# Autodesk Inventor assembly: printer
(part 3 of 3)
- Mate:775: CSN 02 1702 B B 4,3:170 ↔ ISO 4762 M4 x 20:78
- Mate:776: CSN 02 1702 B B 4,3:169 ↔ ISO 4762 M4 x 20:79
- Mate:777: CSN 02 1702 B B 4,3:167 ↔ ISO 4762 M4 x 20:81
- Mate:778: CSN 02 1702 B B 4,3:168 ↔ ISO 4762 M4 x 20:80
- Mate:779: CSN 02 1702 B B 4,3:171 ↔ DIN EN ISO 7040 M4:83
- Mate:780: ISO 4762 M4 x 20:77 ↔ DIN EN ISO 7040 M4:83
- Mate:781: CSN 02 1702 B B 4,3:172 ↔ DIN EN ISO 7040 M4:82
- Mate:782: ISO 4762 M4 x 20:76 ↔ DIN EN ISO 7040 M4:82
- Mate:783: CSN 02 1702 B B 4,3:173 ↔ DIN EN ISO 7040 M4:81
- Mate:784: ISO 4762 M4 x 20:75 ↔ DIN EN ISO 7040 M4:81
- Mate:785: CSN 02 1702 B B 4,3:174 ↔ DIN EN ISO 7040 M4:80
- Mate:786: ISO 4762 M4 x 20:74 ↔ DIN EN ISO 7040 M4:80
- Mate:787: CSN 02 1702 B B 4,3:170 ↔ DIN EN ISO 7040 M4:84
- Mate:788: ISO 4762 M4 x 20:78 ↔ DIN EN ISO 7040 M4:84
- Mate:789: CSN 02 1702 B B 4,3:169 ↔ DIN EN ISO 7040 M4:87
- Mate:790: ISO 4762 M4 x 20:79 ↔ DIN EN ISO 7040 M4:87
- Mate:791: CSN 02 1702 B B 4,3:168 ↔ DIN EN ISO 7040 M4:86
- Mate:792: ISO 4762 M4 x 20:80 ↔ DIN EN ISO 7040 M4:86
- Mate:793: CSN 02 1702 B B 4,3:167 ↔ DIN EN ISO 7040 M4:85
- Mate:794: ISO 4762 M4 x 20:81 ↔ DIN EN ISO 7040 M4:85
- Mate:795: brace_right:1 ↔ IEC inlet:1
- Mate:796: brace_right:1 ↔ IEC inlet:1
- Mate:797: brace_right:1 ↔ IEC inlet:1
- Insert:159: IEC inlet:1 ↔ Cross Recessed Flat Countersunk Head Tapping Screw - Type AB - Type IA - Metric 2,9 x 1 x 8:1
- Insert:160: IEC inlet:1 ↔ Cross Recessed Flat Countersunk Head Tapping Screw - Type AB - Type IA - Metric 2,9 x 1 x 8:2
- Mate:801: back:1 ↔ PC Fan:1
- Mate:802: back:1 ↔ PC Fan:1
- Mate:803: back:1 ↔ PC Fan:1
- Mate:804 (3 mm): back:1 ↔ User Library-Fan Guard:1
- Tangent:3: back:1 ↔ User Library-Fan Guard:1
- Tangent:4: back:1 ↔ User Library-Fan Guard:1
- Insert:161 (0.2 mm): back:1 ↔ Screw F-Z GOST R ISO 7050-93 ST3.5x13-F-Z:1
- Insert:162 (0.2 mm): back:1 ↔ Screw F-Z GOST R ISO 7050-93 ST3.5x13-F-Z:2
- Insert:163 (0.2 mm): back:1 ↔ Screw F-Z GOST R ISO 7050-93 ST3.5x13-F-Z:3
- Insert:164 (0.2 mm): back:1 ↔ Screw F-Z GOST R ISO 7050-93 ST3.5x13-F-Z:4
- Mate:805: frame:1 ↔ z_axis_top:1
- Mate:806: frame:1 ↔ z_axis_top:1
- Mate:807: frame:1 ↔ z_axis_top:1
- Mate:808: z_axis_top:1 ↔ rope_mount_b:1
- Flush:15 (3 mm): z_axis_top:1 ↔ rope_mount_b:1
- Flush:16: z_axis_top:1 ↔ rope_mount_b:1
- Mate:809: z_axis_top:1 ↔ rope_mount_a:1
- Flush:17 (3 mm): z_axis_top:1 ↔ rope_mount_a:1
- Flush:18: z_axis_top:1 ↔ rope_mount_a:1
- Mate:810: rope_mount_b:1 ↔ rope_mount_holder:1
- Mate:811: rope_mount_b:1 ↔ rope_mount_holder:1
- Mate:812: rope_mount_b:1 ↔ rope_mount_holder:1
- Mate:813: frame:1 ↔ z_axis_top:2
- Mate:814: frame:1 ↔ z_axis_top:2
- Mate:815: frame:1 ↔ z_axis_top:2
- Mate:816: z_axis_top:2 ↔ rope_mount_a:2
- Mate:817: z_axis_top:2 ↔ rope_mount_a:2
- Flush:19: z_axis_top:2 ↔ rope_mount_a:2
- Mate:818: z_axis_top:2 ↔ rope_mount_b:2
- Mate:819: z_axis_top:2 ↔ rope_mount_b:2
- Mate:820: z_axis_top:2 ↔ rope_mount_b:2
- Mate:821: z_axis_top:1 ↔ z_axis_top_cap:1
- Mate:822: z_axis_top:1 ↔ z_axis_top_cap:1
- Mate:823: z_axis_top:1 ↔ z_axis_top_cap:1
- Mate:824: z_axis_top:2 ↔ z_axis_top_cap:2
- Mate:825: z_axis_top:2 ↔ z_axis_top_cap:2
- Mate:826: z_axis_top:2 ↔ z_axis_top_cap:2
- Mate:827: rope_mount_b:2 ↔ rope_mount_holder:2
- Mate:828: rope_mount_b:2 ↔ rope_mount_holder:2
- Mate:829: rope_mount_b:2 ↔ rope_mount_holder:2
- Mate:830: z_axis_top_cap:1 ↔ CSN 02 1702 B B 4,3:193
- Mate:831: z_axis_top_cap:1 ↔ CSN 02 1702 B B 4,3:194
- Mate:832: z_axis_top_cap:1 ↔ CSN 02 1702 B B 4,3:194
- Mate:833: z_axis_top_cap:1 ↔ CSN 02 1702 B B 4,3:193
- Mate:834: z_axis_top:1 ↔ CSN 02 1702 B B 4,3:192
- Mate:835: rope_mount_holder:1 ↔ CSN 02 1702 B B 4,3:191
- Mate:836: rope_mount_holder:1 ↔ CSN 02 1702 B B 4,3:189
- Mate:837: rope_mount_holder:1 ↔ CSN 02 1702 B B 4,3:191
- Mate:838: rope_mount_holder:1 ↔ CSN 02 1702 B B 4,3:189
- Mate:839: z_axis_top:1 ↔ CSN 02 1702 B B 4,3:192
- Mate:840: z_axis_top:2 ↔ CSN 02 1702 B B 4,3:183
- Mate:841: z_axis_top:2 ↔ CSN 02 1702 B B 4,3:183
- Mate:842: z_axis_top_cap:2 ↔ CSN 02 1702 B B 4,3:182
- Mate:843: z_axis_top_cap:2 ↔ CSN 02 1702 B B 4,3:184
- Mate:844: z_axis_top_cap:2 ↔ CSN 02 1702 B B 4,3:184
- Mate:845: z_axis_top_cap:2 ↔ CSN 02 1702 B B 4,3:182
- Mate:846: rope_mount_holder:2 ↔ CSN 02 1702 B B 4,3:181
- Mate:847: rope_mount_holder:2 ↔ CSN 02 1702 B B 4,3:180
- Mate:848: rope_mount_holder:2 ↔ CSN 02 1702 B B 4,3:181
- Mate:849: rope_mount_holder:2 ↔ CSN 02 1702 B B 4,3:180
- Insert:165: CSN 02 1702 B B 4,3:194 ↔ ISO 4762 M4 x 20:85
- Insert:166: CSN 02 1702 B B 4,3:193 ↔ ISO 4762 M4 x 20:86
- Insert:167: CSN 02 1702 B B 4,3:192 ↔ ISO 4762 M4 x 20:87
- Insert:168: CSN 02 1702 B B 4,3:182 ↔ ISO 4762 M4 x 20:84
- Insert:169: CSN 02 1702 B B 4,3:184 ↔ ISO 4762 M4 x 20:83
- Insert:170: CSN 02 1702 B B 4,3:183 ↔ ISO 4762 M4 x 20:82
- Insert:171: CSN 02 1702 B B 4,3:181 ↔ ISO 4762 M4 x 35:2
- Insert:172: CSN 02 1702 B B 4,3:180 ↔ ISO 4762 M4 x 35:1
- Insert:173: CSN 02 1702 B B 4,3:191 ↔ ISO 4762 M4 x 35:3
- Insert:174: CSN 02 1702 B B 4,3:189 ↔ ISO 4762 M4 x 35:4
- Mate:850: brace_right:1 ↔ CSN 02 1702 B B 4,3:179
- Mate:851: CSN 02 1702 B B 4,3:179 ↔ ISO 4762 M4 x 35:1
- Mate:852: frame:1 ↔ CSN 02 1702 B B 4,3:178
- Mate:853: CSN 02 1702 B B 4,3:178 ↔ ISO 4762 M4 x 35:2
- Mate:854: frame:1 ↔ CSN 02 1702 B B 4,3:177
- Mate:855: CSN 02 1702 B B 4,3:177 ↔ ISO 4762 M4 x 20:82
- Mate:856: z_axis_top:2 ↔ CSN 02 1702 B B 4,3:176
- Mate:857: z_axis_top:2 ↔ CSN 02 1702 B B 4,3:175
- Mate:858: CSN 02 1702 B B 4,3:176 ↔ ISO 4762 M4 x 20:83
- Mate:859: CSN 02 1702 B B 4,3:175 ↔ ISO 4762 M4 x 20:84
- Mate:860: brace_left:1 ↔ CSN 02 1702 B B 4,3:190
- Mate:861: CSN 02 1702 B B 4,3:190 ↔ ISO 4762 M4 x 35:4
- Mate:862: frame:1 ↔ CSN 02 1702 B B 4,3:188
- Mate:863: CSN 02 1702 B B 4,3:188 ↔ ISO 4762 M4 x 35:3
- Mate:864: frame:1 ↔ CSN 02 1702 B B 4,3:187
- Mate:865: CSN 02 1702 B B 4,3:187 ↔ ISO 4762 M4 x 20:87
- Mate:866: z_axis_top:1 ↔ CSN 02 1702 B B 4,3:185
- Mate:867: z_axis_top:1 ↔ CSN 02 1702 B B 4,3:186
- Mate:868: CSN 02 1702 B B 4,3:186 ↔ ISO 4762 M4 x 20:86
- Mate:869: CSN 02 1702 B B 4,3:185 ↔ ISO 4762 M4 x 20:85
- Mate:870: CSN 02 1702 B B 4,3:179 ↔ DIN EN ISO 7040 M4:91
- Mate:871: ISO 4762 M4 x 35:1 ↔ DIN EN ISO 7040 M4:91
- Mate:872: CSN 02 1702 B B 4,3:177 ↔ DIN EN ISO 7040 M4:92
- Mate:873: ISO 4762 M4 x 20:82 ↔ DIN EN ISO 7040 M4:92
- Mate:874: CSN 02 1702 B B 4,3:178 ↔ DIN EN ISO 7040 M4:90
- Mate:875: ISO 4762 M4 x 35:2 ↔ DIN EN ISO 7040 M4:90
- Mate:876: CSN 02 1702 B B 4,3:175 ↔ DIN EN ISO 7040 M4:88
- Mate:877: ISO 4762 M4 x 20:84 ↔ DIN EN ISO 7040 M4:88
- Mate:878: CSN 02 1702 B B 4,3:176 ↔ DIN EN ISO 7040 M4:89
- Mate:879: ISO 4762 M4 x 20:83 ↔ DIN EN ISO 7040 M4:89
- Mate:880: CSN 02 1702 B B 4,3:190 ↔ DIN EN ISO 7040 M4:95
- Mate:881: ISO 4762 M4 x 35:4 ↔ DIN EN ISO 7040 M4:95
- Mate:882: CSN 02 1702 B B 4,3:188 ↔ DIN EN ISO 7040 M4:93
- Mate:883: ISO 4762 M4 x 35:3 ↔ DIN EN ISO 7040 M4:93
- Mate:884: CSN 02 1702 B B 4,3:187 ↔ DIN EN ISO 7040 M4:94
- Mate:885: ISO 4762 M4 x 20:87 ↔ DIN EN ISO 7040 M4:94
- Mate:886: CSN 02 1702 B B 4,3:185 ↔ DIN EN ISO 7040 M4:96
- Mate:887: ISO 4762 M4 x 20:85 ↔ DIN EN ISO 7040 M4:96
- Mate:888: CSN 02 1702 B B 4,3:186 ↔ DIN EN ISO 7040 M4:97
- Mate:889: ISO 4762 M4 x 20:86 ↔ DIN EN ISO 7040 M4:97
- Mate:890: CSN 02 1702 B B 8,4:7 ↔ CSN 02 1702 B B 8,4:8
- Mate:891: CSN 02 1702 B B 8,4:7 ↔ CSN 02 1702 B B 8,4:8
- Mate:892: CSN 02 1702 B B 8,4:9 ↔ CSN 02 1702 B B 8,4:10
- Mate:893: CSN 02 1702 B B 8,4:9 ↔ CSN 02 1702 B B 8,4:10
- Mate:894: 608RS:2 ↔ CSN 02 1702 B B 8,4:10
- Mate:895: 608RS:2 ↔ CSN 02 1702 B B 8,4:10
- Mate:896: 608RS:2 ↔ CSN 02 1702 B B 8,4:7
- Mate:897: 608RS:2 ↔ CSN 02 1702 B B 8,4:7
- Mate:898: 608RS:2 ↔ rope_pulley:1
- Mate:899: 608RS:2 ↔ rope_pulley:1
- Mate:900: rope_pulley:1 ↔ rope_pulley:2
- Mate:901: rope_pulley:1 ↔ rope_pulley:2
- Mate:902: rope_pulley:1 ↔ rope_pulley:2
- [Mate]: CSN 02 1702 B B 8,4:11 ↔ CSN 02 1702 B B 8,4:12
- [Mate]: CSN 02 1702 B B 8,4:11 ↔ CSN 02 1702 B B 8,4:12
- [Mate]: CSN 02 1702 B B 8,4:13 ↔ CSN 02 1702 B B 8,4:14
- [Mate]: CSN 02 1702 B B 8,4:13 ↔ CSN 02 1702 B B 8,4:14
- [Mate]: 608RS:3 ↔ CSN 02 1702 B B 8,4:14
- [Mate]: 608RS:3 ↔ CSN 02 1702 B B 8,4:14
- [Mate]: 608RS:3 ↔ CSN 02 1702 B B 8,4:11
- [Mate]: 608RS:3 ↔ CSN 02 1702 B B 8,4:11
- [Mate]: 608RS:3 ↔ rope_pulley:3
- [Mate]: 608RS:3 ↔ rope_pulley:3
- [Mate]: rope_pulley:3 ↔ rope_pulley:4
- [Mate]: rope_pulley:3 ↔ rope_pulley:4
- [Mate]: rope_pulley:3 ↔ rope_pulley:4
- [Mate]: CSN 02 1702 B B 8,4:15 ↔ CSN 02 1702 B B 8,4:16
- [Mate]: CSN 02 1702 B B 8,4:15 ↔ CSN 02 1702 B B 8,4:16
- [Mate]: CSN 02 1702 B B 8,4:17 ↔ CSN 02 1702 B B 8,4:18
- [Mate]: CSN 02 1702 B B 8,4:17 ↔ CSN 02 1702 B B 8,4:18
- [Mate]: 608RS:4 ↔ CSN 02 1702 B B 8,4:18
- [Mate]: 608RS:4 ↔ CSN 02 1702 B B 8,4:18
- [Mate]: 608RS:4 ↔ CSN 02 1702 B B 8,4:15
- [Mate]: 608RS:4 ↔ CSN 02 1702 B B 8,4:15
- [Mate]: 608RS:4 ↔ rope_pulley:5
- [Mate]: 608RS:4 ↔ rope_pulley:5
- [Mate]: rope_pulley:5 ↔ rope_pulley:6
- [Mate]: rope_pulley:5 ↔ rope_pulley:6
- [Mate]: rope_pulley:5 ↔ rope_pulley:6
- [Mate]: CSN 02 1702 B B 8,4:19 ↔ CSN 02 1702 B B 8,4:20
- [Mate]: CSN 02 1702 B B 8,4:19 ↔ CSN 02 1702 B B 8,4:20
- [Mate]: CSN 02 1702 B B 8,4:21 ↔ CSN 02 1702 B B 8,4:22
- [Mate]: CSN 02 1702 B B 8,4:21 ↔ CSN 02 1702 B B 8,4:22
- [Mate]: 608RS:5 ↔ CSN 02 1702 B B 8,4:22
- [Mate]: 608RS:5 ↔ CSN 02 1702 B B 8,4:22
- [Mate]: 608RS:5 ↔ CSN 02 1702 B B 8,4:19
- [Mate]: 608RS:5 ↔ CSN 02 1702 B B 8,4:19
- [Mate]: 608RS:5 ↔ rope_pulley:7
- [Mate]: 608RS:5 ↔ rope_pulley:7
- [Mate]: rope_pulley:7 ↔ rope_pulley:8
- [Mate]: rope_pulley:7 ↔ rope_pulley:8
- [Mate]: rope_pulley:7 ↔ rope_pulley:8
- Mate:942: rope_mount_a:2 ↔ CSN 02 1702 B B 8,4:21
- Mate:943: rope_mount_a:2 ↔ CSN 02 1702 B B 8,4:21
- Mate:944: rope_mount_a:2 ↔ CSN 02 1702 B B 8,4:17
- Mate:945: rope_mount_a:2 ↔ CSN 02 1702 B B 8,4:17
- Mate:946: rope_mount_a:1 ↔ CSN 02 1702 B B 8,4:13
- Mate:947: rope_mount_a:1 ↔ CSN 02 1702 B B 8,4:13
- Mate:948: rope_mount_a:1 ↔ CSN 02 1702 B B 8,4:9
- Mate:949: rope_mount_a:1 ↔ CSN 02 1702 B B 8,4:9
- Mate:950: rope_mount_a:1 ↔ CSN 02 1702 B B 8,4:29
- Mate:951: rope_mount_a:1 ↔ CSN 02 1702 B B 8,4:30
- Mate:952: rope_mount_a:2 ↔ CSN 02 1702 B B 8,4:27
- Mate:953: rope_mount_a:2 ↔ CSN 02 1702 B B 8,4:28
- Mate:954: rope_mount_a:1 ↔ CSN 02 1702 B B 8,4:30
- Mate:955: rope_mount_a:1 ↔ CSN 02 1702 B B 8,4:29
- Mate:956: rope_mount_a:2 ↔ CSN 02 1702 B B 8,4:28
- Mate:957: rope_mount_a:2 ↔ CSN 02 1702 B B 8,4:27
- Insert:175: CSN 02 1702 B B 8,4:29 ↔ ISO 4762 M8 x 40:2
- Insert:176: CSN 02 1702 B B 8,4:30 ↔ ISO 4762 M8 x 40:3
- Insert:177: CSN 02 1702 B B 8,4:27 ↔ ISO 4762 M8 x 40:4
- Insert:178: CSN 02 1702 B B 8,4:28 ↔ ISO 4762 M8 x 40:5
- Mate:958: rope_mount_b:2 ↔ CSN 02 1702 B B 8,4:26
- Mate:959: CSN 02 1702 B B 8,4:26 ↔ ISO 4762 M8 x 40:5
- Mate:960: rope_mount_b:2 ↔ CSN 02 1702 B B 8,4:25
- Mate:961: CSN 02 1702 B B 8,4:25 ↔ ISO 4762 M8 x 40:4
- Mate:962: rope_mount_b:1 ↔ CSN 02 1702 B B 8,4:23
- Mate:963: CSN 02 1702 B B 8,4:23 ↔ ISO 4762 M8 x 40:3
- Mate:964: rope_mount_b:1 ↔ CSN 02 1702 B B 8,4:24
- Mate:965: CSN 02 1702 B B 8,4:24 ↔ ISO 4762 M8 x 40:2
- Mate:966: CSN 02 1702 B B 8,4:23 ↔ DIN EN ISO 7040 M8:5
- Mate:967: ISO 4762 M8 x 40:3 ↔ DIN EN ISO 7040 M8:5
- Mate:968: CSN 02 1702 B B 8,4:24 ↔ DIN EN ISO 7040 M8:4
- Mate:969: ISO 4762 M8 x 40:2 ↔ DIN EN ISO 7040 M8:4
- Mate:970: CSN 02 1702 B B 8,4:25 ↔ DIN EN ISO 7040 M8:2
- Mate:971: ISO 4762 M8 x 40:4 ↔ DIN EN ISO 7040 M8:2
- Mate:972: CSN 02 1702 B B 8,4:26 ↔ DIN EN ISO 7040 M8:3
- Mate:973: ISO 4762 M8 x 40:5 ↔ DIN EN ISO 7040 M8:3
- Flush:20: frame:1 ↔ Coffee Mug:1
- Flush:21 (-100 mm): brace_left:1 ↔ Coffee Mug:1
- Flush:22 (100 mm): front:1 ↔ Coffee Mug:1
## Named parameters: d524_d163 = 0 mm, d525_d164 = 0 deg, d526_d165 = 36 deg, d527_d166 = 0 deg, d83_d80 = 0 deg, d84_d81 = 36 deg, d85_d82 = 0 deg, d86_d76 = 0 deg, d87_d77 = 36 deg, d88_d78 = 0 deg, d89_d79 = 0 mm, d90_d75 = 0 mm, d536_d91 = 0 mm, d537_d92 = 0 deg, d538_d93 = 36 deg, d539_d94 = 0 deg, d95_d80 = 0 deg, d96_d81 = 36 deg, d97_d82 = 0 deg, d98_d83_d80 = 0 deg, d99_d84_d81 = 36 deg, d100_d85_d82 = 0 deg, d101_d86_d76 = 0 deg, d102_d87_d77 = 36 deg, d103_d88_d78 = 0 deg, d104_d89_d79 = 0 mm, d105_d90_d75 = 0 mm, d106_d91 = 0 mm, d107_d92 = 0 deg, d108_d93 = 36 deg, d109_d94 = 0 deg, d110_d76 = 0 deg, d111_d77 = 36 deg, d112_d78 = 0 deg, d113_d79 = 0 mm, d114_d75 = 0 mm, d560_d115 = 0 mm, d561_d116 = 0 deg, d562_d117 = 36 deg, d563_d118 = 0 deg, d119_d115 = 0 mm, d120_d116 = 0 deg, d121_d117 = 36 deg, d122_d118 = 0 deg, d123_d80 = 0 deg, d124_d81 = 36 deg, d125_d82 = 0 deg, d126_d83_d80 = 0 deg, d127_d84_d81 = 36 deg, d128_d85_d82 = 0 deg, d129_d86_d76 = 0 deg, d130_d87_d77 = 36 deg, d131_d88_d78 = 0 deg, d132_d89_d79 = 0 mm, d133_d90_d75 = 0 mm, d134_d91 = 0 mm, d135_d92 = 0 deg, d136_d93 = 36 deg, d137_d94 = 0 deg, d153_d110_d76 = 0 deg, d154_d111_d77 = 36 deg, d155_d112_d78 = 0 deg, d157_d114_d75 = 0 mm, d158_d76 = 0 deg, d159_d77 = 36 deg, d160_d78 = 0 deg, d161_d79 = 0 mm, d162_d75 = 0 mm, d608_d75 = 0 mm, d609_d76 = 0 deg, d610_d77 = 36 deg, d611_d78 = 0 deg, d612_d79 = 0 mm, d613_d80 = 0 deg, d614_d81 = 36 deg, d615_d82 = 0 deg, d632_d163 = 0 mm, d633_d164 = 0 deg, d634_d165 = 36 deg, d635_d166 = 0 deg, d636_d83_d80 = 0 deg, d637_d84_d81 = 36 deg, d638_d85_d82 = 0 deg, d639_d86_d76 = 0 deg, d640_d87_d77 = 36 deg, d641_d88_d78 = 0 deg, d642_d89_d79 = 0 mm, d643_d90_d75 = 0 mm, d644_d91 = 0 mm, d645_d92 = 0 deg, d646_d93 = 36 deg, d647_d94 = 0 deg, d648_d95_d80 = 0 deg, d649_d96_d81 = 36 deg, d650_d97_d82 = 0 deg, d651_d98_d83_d80 = 0 deg, d652_d99_d84_d81 = 36 deg, d653_d100_d85_d82 = 0 deg, d654_d101_d86_d76 = 0 deg, d655_d102_d87_d77 = 36 deg, d656_d103_d88_d78 = 0 deg, d657_d104_d89_d79 = 0 mm, d658_d105_d90_d75 = 0 mm, d659_d106_d91 = 0 mm, d660_d107_d92 = 0 deg, d661_d108_d93 = 36 deg, d662_d109_d94 = 0 deg, d663_d110_d76 = 0 deg, d664_d111_d77 = 36 deg, d665_d112_d78 = 0 deg, d666_d113_d79 = 0 mm, d667_d114_d75 = 0 mm, d668_d115 = 0 mm, d669_d116 = 0 deg, d670_d117 = 36 deg, d671_d118 = 0 deg, d672_d119_d115 = 0 mm, d673_d120_d116 = 0 deg, d674_d121_d117 = 36 deg, d675_d122_d118 = 0 deg, d676_d123_d80 = 0 deg, d677_d124_d81 = 36 deg, d678_d125_d82 = 0 deg, d679_d126_d83_d80 = 0 deg, d680_d127_d84_d81 = 36 deg, d681_d128_d85_d82 = 0 deg, d682_d129_d86_d76 = 0 deg, d683_d130_d87_d77 = 36 deg, d684_d131_d88_d78 = 0 deg, d685_d132_d89_d79 = 0 mm, d686_d133_d90_d75 = 0 mm, d687_d134_d91 = 0 mm, d688_d135_d92 = 0 deg, d689_d136_d93 = 36 deg, d690_d137_d94 = 0 deg, d138_d95_d80 = 0 deg, d139_d96_d81 = 36 deg, d140_d97_d82 = 0 deg, d141_d98_d83_d80 = 0 deg, d142_d99_d84_d81 = 36 deg, d143_d100_d85_d82 = 0 deg, d144_d101_d86_d76 = 0 deg, d145_d102_d87_d77 = 36 deg, d146_d103_d88_d78 = 0 deg, d147_d104_d89_d79 = 0 mm, d148_d105_d90_d75 = 0 mm, d149_d106_d91 = 0 mm, d150_d107_d92 = 0 deg, d151_d108_d93 = 36 deg, d152_d109_d94 = 0 deg, d706_d153_d110_d76 = 0 deg, d707_d154_d111_d77 = 36 deg, d708_d155_d112_d78 = 0 deg, d156_d113_d79 = 0 mm, d710_d157_d114_d75 = 0 mm, d711_d158_d76 = 0 deg, d712_d159_d77 = 36 deg, d713_d160_d78 = 0 deg, d714_d161_d79 = 0 mm, d715_d162_d75 = 0 mm, d720_d79 = 0 mm, d721_d80 = 0 deg, d722_d81 = 36 deg, d723_d82 = 0 deg, d1387_d1378 = 0 mm, d1388_d1379 = 0 mm, d1389_d1380 = 0 mm, d1390_d1381 = 0 mm, d1391_d1382 = 0 mm, d1392_d1383 = 0 mm, d1393_d1384 = 0 mm, d1394_d1385 = 0 mm, d1395_d1386 = 0 mm, d1396_d1374 = 0 mm, d1397_d1375 = 0 mm, d1398_d1376 = 0 mm, d1399_d1377 = 0 mm, d1400_d1378 = 0 mm, d1401_d1379 = 0 mm, d1402_d1380 = 0 mm, d1403_d1381 = 0 mm, d1404_d1382 = 0 mm, d1405_d1383 = 0 mm, d1406_d1384 = 0 mm, d1407_d1385 = 0 mm, d1408_d1386 = 0 mm, d1409_d1374 = 0 mm, d1410_d1375 = 0 mm, d1411_d1376 = 0 mm, d1412_d1377 = 0 mm, d1413_d1378 = 0 mm, d1414_d1379 = 0 mm, d1415_d1380 = 0 mm, d1416_d1381 = 0 mm, d1417_d1382 = 0 mm, d1418_d1383 = 0 mm, d1419_d1384 = 0 mm, d1420_d1385 = 0 mm, d1421_d1386 = 0 mm, d1422_d1374 = 0 mm, d1423_d1375 = 0 mm, d1424_d1376 = 0 mm, d1425_d1377 = 0 mm
